# Autodesk Inventor assembly: move_straight
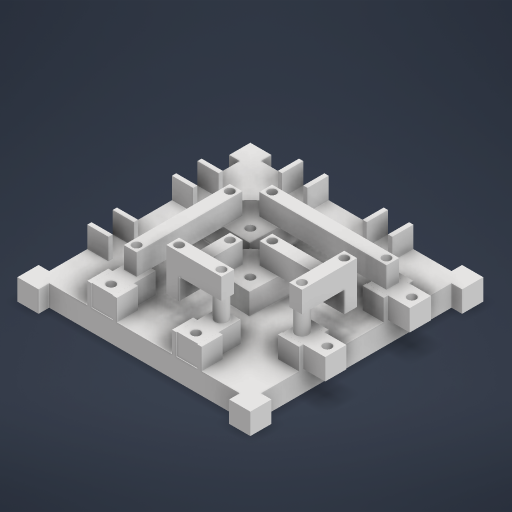
[picture p0: Inventor's stored thumbnail of the model, 512x512]
Saved by Autodesk Inventor 2024.3 (Build 283343000, 343)
## iProperties
Created: 2024-09-29
Part Number: move_straight
Document SubType Name: Assembly
Designer: sam
Author: sam
## Documents named in this file (10)
- N:\Cad\computer\gates\move_left.iam
- N:\Cad\computer\gates\base.ipt
- N:\Cad\computer\gates\block.ipt
- N:\Cad\computer\gates\bellcrank.ipt
- N:\Cad\computer\gates\arm_bellcrank.ipt
- N:\Cad\computer\gates\arm_bellcrank_small.ipt
- N:\Cad\computer\gates\larm_bellcrank.ipt
- N:\Cad\computer\gates\larm_bellcrank_small.ipt
- N:\Cad\computer\gates\spacer_small.ipt
- N:\Cad\computer\gates\bar_bellcrank.ipt
## Components (15 placed, 9 different names)
1. base:1 — Mate:2, Mate:4, Mate:5, Mate:6, Mate:11, Mate:12, Mate:13, Mate:14, Mate:15, Mate:16, Mate:17, Mate:18
2. block:1 — Mate:2, Mate:6, Mate:23, Mate:27
3. block:4 — Mate:4, Mate:5, Mate:19, Mate:21, Flush:1
4. spacer_small:1 — Mate:19, Mate:21, Mate:31, Mate:32
5. bar_bellcrank:1 — Mate:31, Flush:1, Mate:32, Mate:39, Mate:40
6. larm_bellcrank:1 — Mate:39, Mate:40, Mate:41, Mate:42
7. bellcrank:1 — Mate:11, Mate:13, Mate:36, Mate:38, Mate:41, Mate:42
8. arm_bellcrank:1 — Mate:23, Mate:24, Mate:27, Mate:30
9. arm_bellcrank_small:1 — Mate:25, Mate:26, Mate:28, Mate:29
10. larm_bellcrank_small:1 — Mate:35, Mate:36, Mate:37, Mate:38
11. bellcrank:2 — Mate:12, Mate:14, Mate:24, Mate:25, Mate:28, Mate:30
12. bar_bellcrank:2 — Mate:33, Mate:34, Mate:35, Mate:37, Flush:2
13. spacer_small:2 — Mate:20, Mate:22, Mate:33, Mate:34
14. block:6 — Mate:16, Mate:18, Mate:26, Mate:29
15. block:7 — Mate:15, Mate:17, Mate:20, Mate:22, Flush:2
## Relationships (38: Mate 36, Flush 2)
- Mate:2: base:1 ↔ block:1
- Mate:4: base:1 ↔ block:4
- Mate:5: base:1 ↔ block:4
- Mate:6: base:1 ↔ block:1
- Mate:11: base:1 ↔ bellcrank:1
- Mate:12: base:1 ↔ bellcrank:2
- Mate:13: base:1 ↔ bellcrank:1
- Mate:14: base:1 ↔ bellcrank:2
- Mate:15: base:1 ↔ block:7
- Mate:16: base:1 ↔ block:6
- Mate:17: base:1 ↔ block:7
- Mate:18: base:1 ↔ block:6
- Mate:19: block:4 ↔ spacer_small:1
- Mate:20: spacer_small:2 ↔ block:7
- Mate:21: block:4 ↔ spacer_small:1
- Mate:22: spacer_small:2 ↔ block:7
- Mate:23: block:1 ↔ arm_bellcrank:1
- Mate:24: arm_bellcrank:1 ↔ bellcrank:2
- Mate:25: arm_bellcrank_small:1 ↔ bellcrank:2
- Mate:26: arm_bellcrank_small:1 ↔ block:6
- Mate:27: block:1 ↔ arm_bellcrank:1
- Mate:28: arm_bellcrank_small:1 ↔ bellcrank:2
- Mate:29: arm_bellcrank_small:1 ↔ block:6
- Mate:30: arm_bellcrank:1 ↔ bellcrank:2
- Mate:31: spacer_small:1 ↔ bar_bellcrank:1
- Flush:1 (1 mm): block:4 ↔ bar_bellcrank:1
- Mate:32: spacer_small:1 ↔ bar_bellcrank:1
- Mate:33: bar_bellcrank:2 ↔ spacer_small:2
- Mate:34: bar_bellcrank:2 ↔ spacer_small:2
- Mate:35: larm_bellcrank_small:1 ↔ bar_bellcrank:2
- Mate:36: bellcrank:1 ↔ larm_bellcrank_small:1
- Mate:37: larm_bellcrank_small:1 ↔ bar_bellcrank:2
- Mate:38: bellcrank:1 ↔ larm_bellcrank_small:1
- Mate:39: bar_bellcrank:1 ↔ larm_bellcrank:1
- Mate:40: bar_bellcrank:1 ↔ larm_bellcrank:1
- Mate:41: larm_bellcrank:1 ↔ bellcrank:1
- Mate:42: larm_bellcrank:1 ↔ bellcrank:1
- Flush:2 (1 mm): bar_bellcrank:2 ↔ block:7
